# Autodesk Inventor assembly: Mecanismo
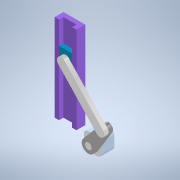
[picture p0: Inventor's stored thumbnail of the model, 180x180]
Saved by Autodesk Inventor 2020.5 (Build 245400000, 400)
## iProperties
Created: 2022-11-03
Part Number: Mecanismo
Document SubType Name: Assembly
Designer: André Aguirre Apolo
Author: André Aguirre Apolo
## iProperties of the stored document Biela.ipt
Created: 2021-10-18
Part Number: Eslabón 3
Material: Steel
Document SubType Name: Modeling
Designer: Usuario
Density: 7.85 g/cm^3
Appearance: Valor por defecto
Mass: 241.553 g
Surface Area: 96.3458 cm^2
Volume: 30.7711 cm^3
Sending System: Autodesk Inventor 2021
Author: Usuario
## iProperties of the stored document Bancada.ipt
Created: 2021-10-18
Part Number: Bancada
Material: Steel
Document SubType Name: Modeling
Designer: Usuario
Density: 7.85 g/cm^3
Appearance: Valor por defecto
Sending System: Autodesk Inventor 2021
Author: Usuario
## iProperties of the stored document Motor.ipt
Created: 2021-10-18
Part Number: MotorEslabon
Material: Steel
Document SubType Name: Modeling
Designer: Usuario
Density: 7.85 g/cm^3
Appearance: Valor por defecto
Sending System: Autodesk Inventor 2021
Author: Usuario
## iProperties of the stored document Manivela.ipt
Created: 2021-10-18
Part Number: Eslabón 2
Material: Stainless Steel
Document SubType Name: Modeling
Designer: Usuario
Density: 8 g/cm^3
Appearance: Valor por defecto
Mass: 146.817 g
Surface Area: 65.052 cm^2
Volume: 18.3522 cm^3
Sending System: Autodesk Inventor 2021
Author: Usuario
## iProperties of the stored document Corredera.ipt
Created: 2021-10-18
Part Number: Corredera
Material: Stainless Steel
Document SubType Name: Modeling
Designer: Usuario
Density: 8 g/cm^3
Appearance: Valor por defecto
Mass: 89.7168 g
Surface Area: 39.5708 cm^2
Volume: 11.2146 cm^3
Sending System: Autodesk Inventor 2021
Author: Usuario
## Documents named in this file (11)
- C:\Users\André Aguirre Apolo\Desktop\ESPOL\PAO2, 2022\Diseño y simulacion de maquinas\Teorico\Mecanismo\Mecanismo.iam
- **C:\Users\André Aguirre Apolo\Desktop\ESPOL\PAO2, 2022\Diseño y simulacion de maquinas\Teorico\Mecanismo\Mecanismo.iam*LocalDocs*xAaaaqqcaAaaaaaaaAaaaqxf2Qb*Motor.ipt
- **C:\Users\André Aguirre Apolo\Desktop\ESPOL\PAO2, 2022\Diseño y simulacion de maquinas\Teorico\Mecanismo\Mecanismo.iam*LocalDocs*xAaaaqbaaAaaaaaaaAaaaqe0yTf*Manivela.ipt
- **C:\Users\André Aguirre Apolo\Desktop\ESPOL\PAO2, 2022\Diseño y simulacion de maquinas\Teorico\Mecanismo\Mecanismo.iam*LocalDocs*xAaaaasbaAaaaaaaaAaaaqwpaSe*Biela.ipt
- **C:\Users\André Aguirre Apolo\Desktop\ESPOL\PAO2, 2022\Diseño y simulacion de maquinas\Teorico\Mecanismo\Mecanismo.iam*LocalDocs*xAaaaqvdaAaaaaaaaAaaaqbjsLd*Corredera.ipt
- **C:\Users\André Aguirre Apolo\Desktop\ESPOL\PAO2, 2022\Diseño y simulacion de maquinas\Teorico\Mecanismo\Mecanismo.iam*LocalDocs*xAaaaagbaAaaaaaaaAaaaqpb11g*Bancada.ipt
- C:\Users\André Aguirre Apolo\Desktop\ESPOL\PAO2, 2022\Diseño y simulacion de maquinas\Teorico\Mecanismo\Motor.ipt
- C:\Users\André Aguirre Apolo\Desktop\ESPOL\PAO2, 2022\Diseño y simulacion de maquinas\Teorico\Mecanismo\Manivela.ipt
- C:\Users\André Aguirre Apolo\Desktop\ESPOL\PAO2, 2022\Diseño y simulacion de maquinas\Teorico\Mecanismo\Biela.ipt
- C:\Users\André Aguirre Apolo\Desktop\ESPOL\PAO2, 2022\Diseño y simulacion de maquinas\Teorico\Mecanismo\Corredera.ipt
- C:\Users\André Aguirre Apolo\Desktop\ESPOL\PAO2, 2022\Diseño y simulacion de maquinas\Teorico\Mecanismo\Bancada.ipt
## Components (5 placed, 5 different names)
1. Motor:1 — Nivelación:1, Insertar:3
2. Manivela:1 — Insertar:3, Insertar:4
3. Biela:1 — Insertar:1, Insertar:4
4. Corredera:1 — Coincidencia:1, Insertar:1
5. Bancada:1 — Nivelación:1, Coincidencia:1
## Relationships (5: Insert 3, Flush 1, Mate 1)
- Nivelación:1 [Flush] (52 mm): Motor:1 ↔ Bancada:1
- Coincidencia:1 [Mate]: Corredera:1 ↔ Bancada:1
- Insertar:1: Biela:1 ↔ Corredera:1
- Insertar:3: Motor:1 ↔ Manivela:1
- Insertar:4: Manivela:1 ↔ Biela:1
